# Autodesk Inventor assembly: Assembly1
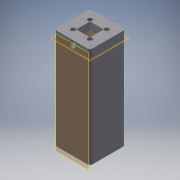
[picture p0: Inventor's stored thumbnail of the model, 180x180]
Saved by Autodesk Inventor 2019.3 (Build 233278000, 278)
## iProperties
Created: 2019-07-14
Part Number: Assembly1
Document SubType Name: Assembly
Designer: mark
Author: mark
## Documents named in this file (3)
- D:\git\photometric-leds\Mechanical\Assembly1.iam
- D:\git\photometric-leds\Mechanical\WeightHolder.ipt
- D:\git\photometric-leds\Mechanical\WeightCap.ipt
## Components (2 placed, 2 different names)
1. WeightHolder:1 — Flush:1, Flush:2, Flush:3
2. WeightCap:1 — Flush:1, Flush:2, Flush:3
## Relationships (3: Flush 3)
- Flush:1: WeightHolder:1 ↔ WeightCap:1
- Flush:2: WeightHolder:1 ↔ WeightCap:1
- Flush:3: WeightHolder:1 ↔ WeightCap:1
